# Autodesk Inventor assembly: brazoRobot
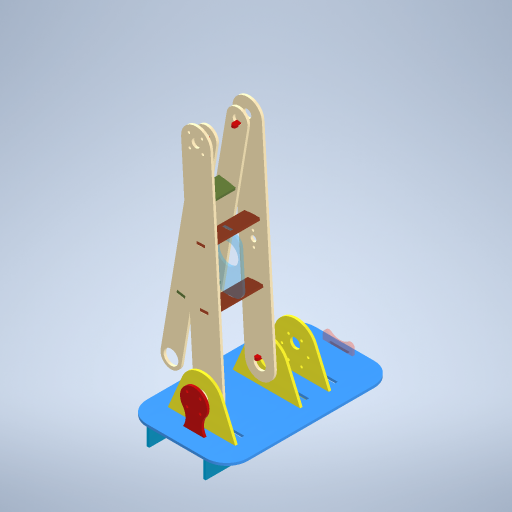
[picture p0: Inventor's stored thumbnail of the model, 512x512]
Saved by Autodesk Inventor 2024.3 (Build 283343000, 343)
## iProperties
Created: 2024-05-14
Part Number: brazoRobot
Document SubType Name: Assembly
Designer: USUARIO
Author: USUARIO
## Documents named in this file (19)
- D:\USUARIO\Documents\Universidad Andres\2024-1\servos\brazoRobot.iam
- D:\USUARIO\Documents\Universidad Andres\2024-1\servos\Base1.ipt
- D:\USUARIO\Documents\Universidad Andres\2024-1\servos\baseSoporte.ipt
- D:\USUARIO\Documents\Universidad Andres\2024-1\servos\brazo1.ipt
- D:\USUARIO\Documents\Universidad Andres\2024-1\servos\unionBrazos1.ipt
- D:\USUARIO\Documents\Universidad Andres\2024-1\servos\unionBrazos.ipt
- D:\USUARIO\Documents\Universidad Andres\2024-1\servos\motor6kg.ipt
- D:\USUARIO\Documents\Universidad Andres\2024-1\servos\brazo2.ipt
- D:\USUARIO\Documents\Universidad Andres\2024-1\servos\soporteM6kg.ipt
- D:\USUARIO\Documents\Universidad Andres\2024-1\servos\eje1.ipt
- D:\USUARIO\Documents\Universidad Andres\2024-1\servos\brazo3.ipt
- D:\USUARIO\Documents\Universidad Andres\2024-1\servos\eje2.ipt
- D:\USUARIO\Documents\Universidad Andres\2024-1\servos\motor12kg.ipt
- D:\USUARIO\Documents\Universidad Andres\2024-1\servos\baseSoporte2.ipt
- D:\USUARIO\Documents\Universidad Andres\2024-1\servos\baseSoporte3.ipt
- D:\USUARIO\Documents\Universidad Andres\2024-1\servos\soporteMotor12kg.ipt
- D:\USUARIO\Documents\Universidad Andres\2024-1\servos\baseInf.ipt
- D:\USUARIO\Documents\Universidad Andres\2024-1\servos\soporteEncoder.ipt
- D:\USUARIO\Documents\Universidad Andres\2024-1\servos\cuña.ipt
## Components (25 placed, 18 different names)
1. Base1:1 — Flush:17, Mate:3, Mate:6, Mate:33, Flush:7, Mate:34, Flush:8, Mate:37, Flush:9, Mate:39, Mate:40, Mate:41, Mate:46, Mate:47, Flush:12
2. baseSoporte:2 — Flush:17, Mate:3, Mate:6, Mate:50, Mate:53, Mate:69, Mate:70
3. brazo1:1 — Mate:7, Mate:8, Mate:9, Mate:10, Mate:11, Mate:12, Insert:8, Insert:9, Insert:13, Mate:38, Insert:14, Insert:16, Mate:65, Mate:67, Mate:68, Flush:18
4. unionBrazos1:1 — Mate:7, Mate:8, Mate:11, Mate:21, Mate:25, Flush:3
5. unionBrazos1:2 — Mate:9, Mate:10, Mate:12, Flush:1, Mate:22, Mate:65, Mate:26, Mate:66
6. unionBrazos:1 — Mate:29, Flush:5, Mate:30, Flush:6, Mate:32
7. unionBrazos:2 — Mate:27, Flush:4, Mate:62, Mate:63
8. motor6kg:1 — Insert:6
9. brazo2:1 — Insert:6, Mate:21, Mate:25, Flush:3, Mate:66
10. soporteM6kg:1 — Flush:1, Mate:22, Mate:26
11. eje1:1 — Insert:13, Mate:38, Insert:15, Insert:16, Mate:54, Mate:55, Flush:13, Mate:56, Flush:14, Mate:57
12. brazo3:1 — Flush:6, Mate:32, Mate:63
13. brazo3:2 — Insert:8, Mate:27, Flush:4, Mate:29, Flush:5, Mate:30, Insert:14, Mate:62, Mate:64
14. eje2:1 — Insert:9, Mate:58, Flush:15, Mate:59, Mate:60, Mate:61, Flush:16
15. baseSoporte2:1 — Mate:33, Flush:7, Mate:34, Insert:15, Mate:48, Mate:51
16. motor12kg:1 — Insert:11, Insert:12
17. baseSoporte3:1 — Flush:8, Mate:37, Insert:11, Insert:12, Mate:41
18. soporteMotor12kg:1 — Flush:9, Mate:39, Mate:40
19. baseInf:1 — Mate:51, Mate:53, Mate:69
20. baseInf:2 — Mate:48, Mate:50, Mate:70
21. soporteEncoder:1 — Mate:46, Mate:47, Flush:12
22. cuña:1 — Mate:54, Mate:55, Flush:13, Mate:67, Mate:68, Flush:18
23. cuña:2 — Mate:56, Flush:14, Mate:57
24. cuña:3 — Mate:60, Mate:61, Flush:16, Mate:64
25. cuña:4 — Mate:58, Flush:15, Mate:59
## Relationships (70: Mate 46, Flush 15, Insert 9)
- Flush:17: Base1:1 ↔ baseSoporte:2
- Mate:3: Base1:1 ↔ baseSoporte:2
- Mate:6: Base1:1 ↔ baseSoporte:2
- Mate:7: brazo1:1 ↔ unionBrazos1:1
- Mate:8: brazo1:1 ↔ unionBrazos1:1
- Mate:9: brazo1:1 ↔ unionBrazos1:2
- Mate:10: brazo1:1 ↔ unionBrazos1:2
- Mate:11: brazo1:1 ↔ unionBrazos1:1
- Mate:12: brazo1:1 ↔ unionBrazos1:2
- Insert:6: motor6kg:1 ↔ brazo2:1
- Mate:21: unionBrazos1:1 ↔ brazo2:1
- Flush:1: unionBrazos1:2 ↔ soporteM6kg:1
- Mate:22: unionBrazos1:2 ↔ soporteM6kg:1
- Mate:25: unionBrazos1:1 ↔ brazo2:1
- Flush:3: unionBrazos1:1 ↔ brazo2:1
- Mate:26: unionBrazos1:2 ↔ soporteM6kg:1
- Insert:8 (9 mm): brazo1:1 ↔ brazo3:2
- Mate:27: unionBrazos:2 ↔ brazo3:2
- Flush:4: unionBrazos:2 ↔ brazo3:2
- Mate:29: unionBrazos:1 ↔ brazo3:2
- Flush:5: unionBrazos:1 ↔ brazo3:2
- Mate:30: unionBrazos:1 ↔ brazo3:2
- Flush:6: unionBrazos:1 ↔ brazo3:1
- Mate:32: unionBrazos:1 ↔ brazo3:1
- Insert:9 (-7 mm): brazo1:1 ↔ eje2:1
- Mate:33: Base1:1 ↔ baseSoporte2:1
- Flush:7: Base1:1 ↔ baseSoporte2:1
- Mate:34: Base1:1 ↔ baseSoporte2:1
- Flush:8: Base1:1 ↔ baseSoporte3:1
- Mate:37: Base1:1 ↔ baseSoporte3:1
- Insert:11: motor12kg:1 ↔ baseSoporte3:1
- Insert:12: motor12kg:1 ↔ baseSoporte3:1
- Insert:13 (1 mm): brazo1:1 ↔ eje1:1
- Mate:38: brazo1:1 ↔ eje1:1
- Flush:9: Base1:1 ↔ soporteMotor12kg:1
- Mate:39: Base1:1 ↔ soporteMotor12kg:1
- Mate:40: Base1:1 ↔ soporteMotor12kg:1
- Insert:14 (-12 mm): brazo1:1 ↔ brazo3:2
- Insert:15 (5 mm): eje1:1 ↔ baseSoporte2:1
- Insert:16 (-3 mm): brazo1:1 ↔ eje1:1
- Mate:41: Base1:1 ↔ baseSoporte3:1
- Mate:46: Base1:1 ↔ soporteEncoder:1
- Mate:47: Base1:1 ↔ soporteEncoder:1
- Flush:12: Base1:1 ↔ soporteEncoder:1
- Mate:48: baseSoporte2:1 ↔ baseInf:2
- Mate:50: baseSoporte:2 ↔ baseInf:2
- Mate:51: baseSoporte2:1 ↔ baseInf:1
- Mate:53: baseSoporte:2 ↔ baseInf:1
- Mate:54: eje1:1 ↔ cuña:1
- Mate:55: eje1:1 ↔ cuña:1
- Flush:13: eje1:1 ↔ cuña:1
- Mate:56: eje1:1 ↔ cuña:2
- Flush:14: eje1:1 ↔ cuña:2
- Mate:57: eje1:1 ↔ cuña:2
- Mate:58: eje2:1 ↔ cuña:4
- Flush:15: eje2:1 ↔ cuña:4
- Mate:59: eje2:1 ↔ cuña:4
- Mate:60: eje2:1 ↔ cuña:3
- Mate:61: eje2:1 ↔ cuña:3
- Flush:16: eje2:1 ↔ cuña:3
- Mate:62: unionBrazos:2 ↔ brazo3:2
- Mate:63: unionBrazos:2 ↔ brazo3:1
- Mate:64: brazo3:2 ↔ cuña:3
- Mate:65: brazo1:1 ↔ unionBrazos1:2
- Mate:66: unionBrazos1:2 ↔ brazo2:1
- Mate:67: brazo1:1 ↔ cuña:1
- Mate:68: brazo1:1 ↔ cuña:1
- Flush:18: brazo1:1 ↔ cuña:1
- Mate:69: baseSoporte:2 ↔ baseInf:1
- Mate:70: baseSoporte:2 ↔ baseInf:2
